# Autodesk Inventor assembly: right
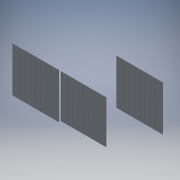
[picture p0: Inventor's stored thumbnail of the model, 180x180]
Saved by Autodesk Inventor 2019 (Build 230136000, 136)
## iProperties
Created: 2018-07-10
Part Number: right
Document SubType Name: Assembly
Designer: User
Author: User
## Documents named in this file (4)
- C:\Users\User\Desktop\Room Model\right.iam
- C:\Users\User\Desktop\Room Model\right_0_0.ipt
- C:\Users\User\Desktop\Room Model\right_0_1.ipt
- C:\Users\User\Desktop\Room Model\right_0_2.ipt
## Components (3 placed, 3 different names)
1. right_0_0:1 — Rigid:1
2. right_0_1:1 — Rigid:1
3. right_0_2:1
## Relationships (1: WeldJoint 1)
- Rigid:1 [WeldJoint] (57.15 mm): right_0_0:1 ↔ right_0_1:1
